# Autodesk Inventor assembly: Setup_1_part_4
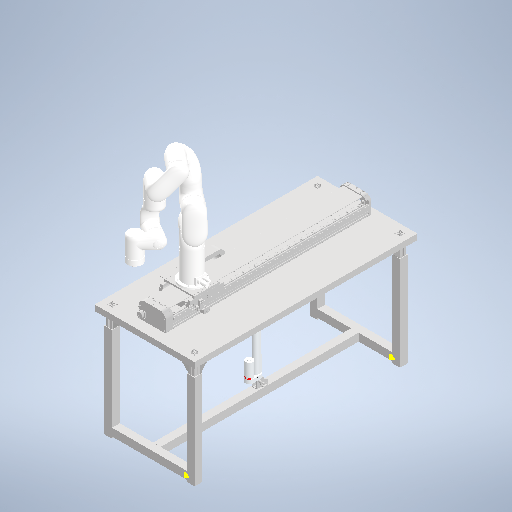
[picture p0: Inventor's stored thumbnail of the model, 512x512]
Saved by Autodesk Inventor 2025 (Build 290162000, 162)
## iProperties
Created: 2024-06-27
Part Number: Setup_1_part_4
Document SubType Name: Assembly
Designer: User
Author: User
## Documents named in this file (15)
- C:\Users\User\OneDrive\Documents\FYP\Inventor_Designs\Setups\Setup_1_part_4.iam
- C:\Users\User\OneDrive\Documents\FYP\Inventor_Designs\Platform\Platform_Arm_2.ipt
- C:\Users\User\OneDrive\Documents\FYP\Inventor_Designs\Metal Profile\Metal Profile 50 cm.ipt
- C:\Users\User\OneDrive\Documents\FYP\Inventor_Designs\Metal Profile\Tube 55 cm.ipt
- C:\Users\User\OneDrive\Documents\FYP\Inventor_Designs\Metal Profile\Tube 40 cm.ipt
- C:\Users\User\OneDrive\Documents\FYP\Inventor_Designs\Metal Profile\Tube 104 cm.ipt
- C:\Users\User\OneDrive\Documents\FYP\Inventor_Designs\Linear Motor\Motor.ipt
- C:\Users\User\OneDrive\Documents\FYP\Inventor_Designs\Designs_Arm\Arm.iam
- C:\Users\User\OneDrive\Documents\FYP\Inventor_Designs\Triangle Bracket\Triangle Bracket.ipt
- C:\Users\User\OneDrive\Documents\FYP\Inventor_Designs\Linear Actuator\300mm Body.ipt
- C:\Users\User\OneDrive\Documents\FYP\Inventor_Designs\Clevis Pin\Celvis Pin.ipt
- C:\Users\User\OneDrive\Documents\FYP\Inventor_Designs\Linear Actuator\300mm Rod.ipt
- C:\Users\User\OneDrive\Documents\FYP\Inventor_Designs\Metal Profile\Metal Profile 104 cm.ipt
- C:\Users\User\OneDrive\Documents\FYP\Inventor_Designs\Metal Profile\Metal Profile 40 cm.ipt
- C:\Users\User\OneDrive\Documents\FYP\Inventor_Designs\L Bracket\L Angle Bracket 30x30.ipt
## Components (31 placed, 14 different names)
1. Platform_Arm_2:1 — Mate:1, Mate:2, Flush:1, Mate:3, Mate:4, Flush:2, Mate:5, Mate:6, Flush:3, Mate:7, Mate:8, Flush:4, Mate:30, Flush:15, Flush:16, Mate:35, Flush:19, Flush:20
2. Metal Profile 50 cm:1 — Mate:1, Mate:2, Flush:1, Mate:23, Mate:24, Mate:43, Flush:29, Flush:30, Flush:31, Flush:32, Mate:44, Flush:33, Mate:47, Flush:36, Mate:59
3. Metal Profile 50 cm:2 — Mate:5, Mate:6, Flush:3, Flush:37, Mate:49, Flush:42, Mate:61
4. Metal Profile 50 cm:3 — Mate:3, Mate:4, Flush:2, Mate:42, Flush:26, Flush:27, Flush:28, Flush:39, Mate:53, Mate:54, Flush:40
5. Metal Profile 50 cm:4 — Mate:7, Mate:8, Flush:4, Mate:45, Flush:34, Flush:35, Flush:38, Mate:51, Mate:57, Flush:41
6. Tube 55 cm:1 — Mate:23, Mate:24, Mate:37, Flush:21, Flush:22
7. Tube 55 cm:2 — Flush:10, Mate:36
8. Tube 104 cm:1 — Flush:10, Flush:14, Mate:32, Flush:17, Mate:38, Flush:23
9. Tube 55 cm:3 — Flush:14, Mate:39, Flush:24, Flush:25
10. Tube 55 cm:4 — Mate:40
11. Motor:1 — Mate:30, Flush:15, Flush:16
12. Arm:1 [sub-assembly]
13. Triangle Bracket:1 — Mate:32, Flush:17
14. 300mm Body:1 — Mate:33, Mate:41
15. Celvis Pin:1
16. 300mm Rod:3 — Mate:33, Mate:34, Mate:41
17. Triangle Bracket:2 — Mate:34, Mate:35, Flush:19, Flush:20
18. Tube 40 cm:1 — Mate:36, Mate:37, Flush:21, Flush:22, Mate:38, Flush:23
19. Tube 40 cm:2 — Mate:39, Mate:40, Flush:24, Flush:25
20. Metal Profile 104 cm:1 — Mate:42, Flush:26, Flush:27, Flush:28, Mate:50, Mate:52
21. Metal Profile 104 cm:2 — Mate:43, Flush:29, Flush:30, Flush:31, Mate:46, Mate:48
22. Metal Profile 40 cm:1 — Flush:32, Mate:44, Flush:33, Mate:55, Mate:58
23. Metal Profile 40 cm:2 — Mate:45, Flush:34, Flush:35, Mate:56, Mate:60
24. L Angle Bracket 30x30:1 — Mate:46, Mate:47, Flush:36
25. L Angle Bracket 30x30:2 — Flush:39, Mate:52, Mate:53
26. L Angle Bracket 30x30:3 — Flush:38, Mate:50, Mate:51
27. L Angle Bracket 30x30:4 — Flush:37, Mate:48, Mate:49
28. L Angle Bracket 30x30:5 — Mate:58, Mate:59
29. L Angle Bracket 30x30:7 — Mate:54, Flush:40, Mate:55
30. L Angle Bracket 30x30:8 — Mate:56, Mate:57, Flush:41
31. L Angle Bracket 30x30:9 — Mate:60, Flush:42, Mate:61
## Relationships (79: Mate 45, Flush 33, Insert 1)
- Mate:1: Platform_Arm_2:1 ↔ Metal Profile 50 cm:1
- Mate:2: Platform_Arm_2:1 ↔ Metal Profile 50 cm:1
- Flush:1: Platform_Arm_2:1 ↔ Metal Profile 50 cm:1
- Mate:3: Platform_Arm_2:1 ↔ Metal Profile 50 cm:3
- Mate:4: Platform_Arm_2:1 ↔ Metal Profile 50 cm:3
- Flush:2: Platform_Arm_2:1 ↔ Metal Profile 50 cm:3
- Mate:5: Platform_Arm_2:1 ↔ Metal Profile 50 cm:2
- Mate:6: Platform_Arm_2:1 ↔ Metal Profile 50 cm:2
- Flush:3: Platform_Arm_2:1 ↔ Metal Profile 50 cm:2
- Mate:7: Platform_Arm_2:1 ↔ Metal Profile 50 cm:4
- Mate:8: Platform_Arm_2:1 ↔ Metal Profile 50 cm:4
- Flush:4: Platform_Arm_2:1 ↔ Metal Profile 50 cm:4
- Flush:10 (215.9 mm): Tube 55 cm:2 ↔ Tube 104 cm:1
- Flush:14 (215.9 mm): Tube 104 cm:1 ↔ Tube 55 cm:3
- Mate:23 (2 mm): Metal Profile 50 cm:1 ↔ Tube 55 cm:1
- Mate:24 (2 mm): Metal Profile 50 cm:1 ↔ Tube 55 cm:1
- [Mate]: Motor:1 ↔ Arm:1
- [Mate]: Motor:1 ↔ Arm:1
- [Mate]: Motor:1 ↔ Arm:1
- Mate:30: Platform_Arm_2:1 ↔ Motor:1
- Flush:15 (200 mm): Platform_Arm_2:1 ↔ Motor:1
- Flush:16 (50 mm): Platform_Arm_2:1 ↔ Motor:1
- [Insert] (-22 mm): Triangle Bracket:1 ↔ 300mm Body:1
- [Mate]: Triangle Bracket:1 ↔ Celvis Pin:1
- Mate:32: Tube 104 cm:1 ↔ Triangle Bracket:1
- Flush:17 (7 mm): Tube 104 cm:1 ↔ Triangle Bracket:1
- Mate:33: 300mm Body:1 ↔ 300mm Rod:3
- Mate:34: 300mm Rod:3 ↔ Triangle Bracket:2
- Mate:35: Platform_Arm_2:1 ↔ Triangle Bracket:2
- Flush:19 (248 mm): Platform_Arm_2:1 ↔ Triangle Bracket:2
- Flush:20 (320 mm): Platform_Arm_2:1 ↔ Triangle Bracket:2
- Mate:36: Tube 55 cm:2 ↔ Tube 40 cm:1
- Mate:37: Tube 55 cm:1 ↔ Tube 40 cm:1
- Flush:21: Tube 55 cm:1 ↔ Tube 40 cm:1
- Flush:22 (10 mm): Tube 55 cm:1 ↔ Tube 40 cm:1
- Mate:38: Tube 104 cm:1 ↔ Tube 40 cm:1
- Flush:23: Tube 104 cm:1 ↔ Tube 40 cm:1
- Mate:39: Tube 55 cm:3 ↔ Tube 40 cm:2
- Mate:40: Tube 55 cm:4 ↔ Tube 40 cm:2
- Flush:24: Tube 55 cm:3 ↔ Tube 40 cm:2
- Flush:25 (10 mm): Tube 55 cm:3 ↔ Tube 40 cm:2
- Mate:41: 300mm Body:1 ↔ 300mm Rod:3
- Mate:42: Metal Profile 50 cm:3 ↔ Metal Profile 104 cm:1
- Flush:26: Metal Profile 50 cm:3 ↔ Metal Profile 104 cm:1
- Flush:27: Metal Profile 50 cm:3 ↔ Metal Profile 104 cm:1
- Flush:28 (30 mm): Metal Profile 50 cm:3 ↔ Metal Profile 104 cm:1
- Mate:43: Metal Profile 50 cm:1 ↔ Metal Profile 104 cm:2
- Flush:29: Metal Profile 50 cm:1 ↔ Metal Profile 104 cm:2
- Flush:30: Metal Profile 50 cm:1 ↔ Metal Profile 104 cm:2
- Flush:31 (30 mm): Metal Profile 50 cm:1 ↔ Metal Profile 104 cm:2
- Flush:32: Metal Profile 50 cm:1 ↔ Metal Profile 40 cm:1
- Mate:44: Metal Profile 50 cm:1 ↔ Metal Profile 40 cm:1
- Flush:33 (30 mm): Metal Profile 50 cm:1 ↔ Metal Profile 40 cm:1
- Mate:45: Metal Profile 50 cm:4 ↔ Metal Profile 40 cm:2
- Flush:34: Metal Profile 50 cm:4 ↔ Metal Profile 40 cm:2
- Flush:35 (30 mm): Metal Profile 50 cm:4 ↔ Metal Profile 40 cm:2
- Mate:46: Metal Profile 104 cm:2 ↔ L Angle Bracket 30x30:1
- Mate:47: Metal Profile 50 cm:1 ↔ L Angle Bracket 30x30:1
- Flush:36: Metal Profile 50 cm:1 ↔ L Angle Bracket 30x30:1
- Flush:37: Metal Profile 50 cm:2 ↔ L Angle Bracket 30x30:4
- Mate:48: Metal Profile 104 cm:2 ↔ L Angle Bracket 30x30:4
- Mate:49: Metal Profile 50 cm:2 ↔ L Angle Bracket 30x30:4
- Flush:38: Metal Profile 50 cm:4 ↔ L Angle Bracket 30x30:3
- Mate:50: Metal Profile 104 cm:1 ↔ L Angle Bracket 30x30:3
- Mate:51: Metal Profile 50 cm:4 ↔ L Angle Bracket 30x30:3
- Flush:39: Metal Profile 50 cm:3 ↔ L Angle Bracket 30x30:2
- Mate:52: Metal Profile 104 cm:1 ↔ L Angle Bracket 30x30:2
- Mate:53: Metal Profile 50 cm:3 ↔ L Angle Bracket 30x30:2
- Mate:54: Metal Profile 50 cm:3 ↔ L Angle Bracket 30x30:7
- Flush:40: Metal Profile 50 cm:3 ↔ L Angle Bracket 30x30:7
- Mate:55: Metal Profile 40 cm:1 ↔ L Angle Bracket 30x30:7
- Mate:56: Metal Profile 40 cm:2 ↔ L Angle Bracket 30x30:8
- Mate:57: Metal Profile 50 cm:4 ↔ L Angle Bracket 30x30:8
- Flush:41: Metal Profile 50 cm:4 ↔ L Angle Bracket 30x30:8
- Mate:58: Metal Profile 40 cm:1 ↔ L Angle Bracket 30x30:5
- Mate:59: Metal Profile 50 cm:1 ↔ L Angle Bracket 30x30:5
- Mate:60: Metal Profile 40 cm:2 ↔ L Angle Bracket 30x30:9
- Flush:42: Metal Profile 50 cm:2 ↔ L Angle Bracket 30x30:9
- Mate:61: Metal Profile 50 cm:2 ↔ L Angle Bracket 30x30:9
